# Autodesk Inventor assembly: Track Design 9-24-19
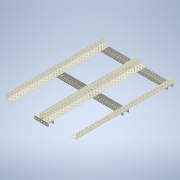
[picture p0: Inventor's stored thumbnail of the model, 180x180]
Saved by Autodesk Inventor 2020 (Build 240168000, 168)
## iProperties
Created: 2019-07-25
Part Number: Track Design 9-24-19
Document SubType Name: Assembly
Designer: Corey
Author: Corey
## Documents named in this file (5)
- C:\Users\Corey\Documents\Tower-Takeover-CAD\Parts\Dual Track.iam
- C:\Users\Corey\Documents\Tower-Takeover-CAD\Parts\Structure\90 Degree Brackets\Aluminum\Aluminum Angle 2x2x35.ipt
- C:\Users\Corey\Documents\Tower-Takeover-CAD\Parts\Cube.iam
- C:\Users\Corey\Documents\Tower-Takeover-CAD\Parts\Structure\C-Channels\Aluminum\2-Wide\Aluminum C-Channel 1x2x1x25.ipt
- C:\Users\Corey\Documents\Tower-Takeover-CAD\Parts\Structure\C-Channels\Aluminum\2-Wide\Aluminum C-Channel 1x2x1x5.ipt
## Components (9 placed, 4 different names)
1. Aluminum Angle 2x2x35:1 — Flush:4, Flush:5, Flush:6, Mate:2, Flush:13, Flush:14
2. Aluminum Angle 2x2x35:2 — Flush:1, Flush:2, Flush:3, Flush:9, Flush:10
3. Aluminum Angle 2x2x35:3 — Flush:1, Flush:2, Flush:4, Mate:1, Flush:11, Flush:12, Mate:3, Flush:15, Flush:16
4. Aluminum Angle 2x2x35:4 — Flush:3, Flush:7, Flush:8
5. Cube:1 [sub-assembly]
6. Cube:2 [sub-assembly]
7. Aluminum C-Channel 1x2x1x25:1 — Mate:2, Flush:13, Flush:14
8. Aluminum C-Channel 1x2x1x25:3 — Mate:1, Flush:5, Flush:6, Flush:7, Flush:8, Flush:9, Flush:10, Flush:11, Flush:12
9. Aluminum C-Channel 1x2x1x5:1 — Mate:3, Flush:15, Flush:16
## Relationships (19: Flush 16, Mate 3)
- Flush:1: Aluminum Angle 2x2x35:2 ↔ Aluminum Angle 2x2x35:3
- Flush:2: Aluminum Angle 2x2x35:2 ↔ Aluminum Angle 2x2x35:3
- Flush:3: Aluminum Angle 2x2x35:2 ↔ Aluminum Angle 2x2x35:4
- Flush:4: Aluminum Angle 2x2x35:1 ↔ Aluminum Angle 2x2x35:3
- Mate:1: Aluminum Angle 2x2x35:3 ↔ Aluminum C-Channel 1x2x1x25:3
- Flush:5: Aluminum Angle 2x2x35:1 ↔ Aluminum C-Channel 1x2x1x25:3
- Flush:6: Aluminum Angle 2x2x35:1 ↔ Aluminum C-Channel 1x2x1x25:3
- Flush:7: Aluminum Angle 2x2x35:4 ↔ Aluminum C-Channel 1x2x1x25:3
- Flush:8: Aluminum Angle 2x2x35:4 ↔ Aluminum C-Channel 1x2x1x25:3
- Flush:9: Aluminum Angle 2x2x35:2 ↔ Aluminum C-Channel 1x2x1x25:3
- Flush:10: Aluminum Angle 2x2x35:2 ↔ Aluminum C-Channel 1x2x1x25:3
- Flush:11: Aluminum Angle 2x2x35:3 ↔ Aluminum C-Channel 1x2x1x25:3
- Flush:12: Aluminum Angle 2x2x35:3 ↔ Aluminum C-Channel 1x2x1x25:3
- Mate:2: Aluminum Angle 2x2x35:1 ↔ Aluminum C-Channel 1x2x1x25:1
- Flush:13: Aluminum Angle 2x2x35:1 ↔ Aluminum C-Channel 1x2x1x25:1
- Flush:14: Aluminum Angle 2x2x35:1 ↔ Aluminum C-Channel 1x2x1x25:1
- Mate:3: Aluminum Angle 2x2x35:3 ↔ Aluminum C-Channel 1x2x1x5:1
- Flush:15: Aluminum Angle 2x2x35:3 ↔ Aluminum C-Channel 1x2x1x5:1
- Flush:16: Aluminum Angle 2x2x35:3 ↔ Aluminum C-Channel 1x2x1x5:1
